# Autodesk Inventor assembly: LeftAndRightPinAttatchments-1111-2020
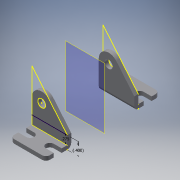
[picture p0: Inventor's stored thumbnail of the model, 180x180]
Saved by Autodesk Inventor 2018 (Build 220112000, 112)
## iProperties
Created: 2020-02-08
Part Number: LeftAndRightPinAttatchments-1111-2020
Document SubType Name: Assembly
Designer: JMHal
Author: JMHal
## Documents named in this file (3)
- E:\PHRC CADD\Resources\Pneumatic Resources\LeftAndRightPinAttatchments-1111-2020.iam
- E:\PHRC CADD\Resources\Pneumatic Resources\LeftPinAtttachments-1111-2019.ipt
- E:\PHRC CADD\Resources\Pneumatic Resources\LeftPinAtttachments-1111-2019_MIR.ipt
## Components (2 placed, 2 different names)
1. LeftPinAtttachments-1111-2019:1 — Flush:1
2. LeftPinAtttachments-1111-2019_MIR:1 — Mate:1
## Relationships (2: Flush 1, Mate 1)
- Flush:1 (25.4 mm): LeftPinAtttachments-1111-2019:1
- Mate:1 (25.4 mm): LeftPinAtttachments-1111-2019_MIR:1
